# Autodesk Inventor assembly: Assembly
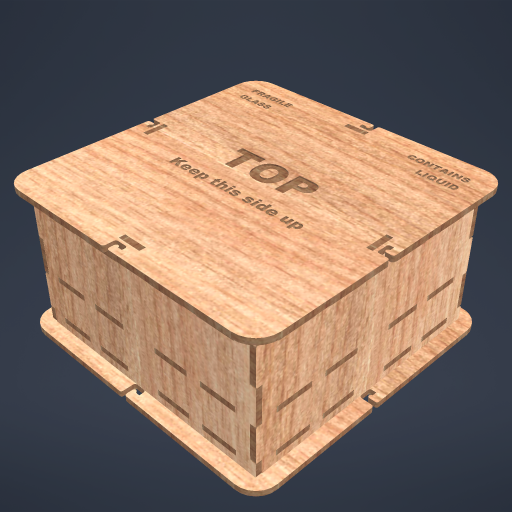
[picture p0: Inventor's stored thumbnail of the model, 512x512]
Saved by Autodesk Inventor 2024.1 (Build 281209000, 209)
## iProperties
Created: 2024-05-23
Part Number: Assembly
Document SubType Name: Assembly
Designer: Tim Jäger
Author: Tim Jäger
## Documents named in this file (7)
- D:\Users\Tim\VUB\Master_Embedded\Master_Thesis\Files3D\TubeHolder_Large\Assembly.iam
- D:\Users\Tim\VUB\Master_Embedded\Master_Thesis\Files3D\TubeHolder_Large\Bottom.ipt
- D:\Users\Tim\VUB\Master_Embedded\Master_Thesis\Files3D\TubeHolder_Large\Side.ipt
- D:\Users\Tim\VUB\Master_Embedded\Master_Thesis\Files3D\TubeHolder_Large\MiddleGrid.ipt
- D:\Users\Tim\VUB\Master_Embedded\Master_Thesis\Files3D\TubeHolder_Large\TopGrid.ipt
- D:\Users\Tim\VUB\Master_Embedded\Master_Thesis\Files3D\TubeHolder_Large\Solid.ipt
- D:\Users\Tim\VUB\Master_Embedded\Master_Thesis\Files3D\TubeHolder_Large\Lid.ipt
## Components (9 placed, 6 different names)
1. Bottom:1 — Mate:1, Mate:2, Mate:3, Mate:4, Mate:5
2. Side:1 — Flush:3, Mate:1, Mate:2, Mate:8, Mate:17, Mate:21
3. Side:2 — Flush:1, Mate:3, Mate:7, Mate:8, Mate:9, Mate:11, Mate:18, Mate:19, Mate:20
4. Side:3 — Flush:1, Flush:2, Mate:4, Mate:6, Mate:7, Mate:9, Mate:13, Mate:16
5. Side:4 — Flush:2, Flush:3, Mate:5, Mate:6, Mate:10, Mate:12, Mate:14, Mate:15
6. MiddleGrid:1 — Mate:11, Mate:17, Mate:18
7. TopGrid:1 — Mate:10, Mate:15, Mate:16
8. Solid:1 — Mate:12, Mate:13, Mate:14
9. Lid:1 — Mate:19, Mate:20, Mate:21
## Relationships (24: Mate 21, Flush 3)
- Flush:1: Side:2 ↔ Side:3
- Flush:2: Side:3 ↔ Side:4
- Flush:3: Side:1 ↔ Side:4
- Mate:1: Bottom:1 ↔ Side:1
- Mate:2: Bottom:1 ↔ Side:1
- Mate:3: Bottom:1 ↔ Side:2
- Mate:4: Bottom:1 ↔ Side:3
- Mate:5: Bottom:1 ↔ Side:4
- Mate:6: Side:3 ↔ Side:4
- Mate:7: Side:2 ↔ Side:3
- Mate:8: Side:1 ↔ Side:2
- Mate:9: Side:2 ↔ Side:3
- Mate:10: Side:4 ↔ TopGrid:1
- Mate:11: Side:2 ↔ MiddleGrid:1
- Mate:12: Side:4 ↔ Solid:1
- Mate:13: Side:3 ↔ Solid:1
- Mate:14: Side:4 ↔ Solid:1
- Mate:15: Side:4 ↔ TopGrid:1
- Mate:16: Side:3 ↔ TopGrid:1
- Mate:17: Side:1 ↔ MiddleGrid:1
- Mate:18: Side:2 ↔ MiddleGrid:1
- Mate:19: Side:2 ↔ Lid:1
- Mate:20: Side:2 ↔ Lid:1
- Mate:21: Side:1 ↔ Lid:1
